# Autodesk Inventor assembly: ラックアンドピニオン
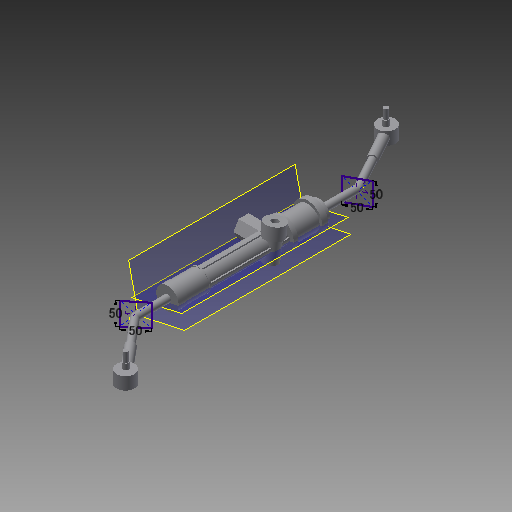
[picture p0: Inventor's stored thumbnail of the model, 512x512]
Saved by Autodesk Inventor 2018 (Build 220112000, 112)
## iProperties
Created: 2017-09-10
Part Number: ラックアンドピニオン
Material: 一般
Document SubType Name: Assembly
Designer: Kenta
Author: Kenta
## Documents named in this file (4)
- C:\Users\Kenta\Documents\workspace\rbbr\cart\ラックアンドピニオン.iam
- C:\Users\Kenta\Documents\workspace\rbbr\cart\らっくあんどぴにおん.ipt
- C:\Users\Kenta\Documents\workspace\rbbr\cart\ラックアンドピニオンの中心棒.ipt
- C:\Users\Kenta\Documents\workspace\rbbr\cart\ラックアンドピニオンの左右の棒.ipt
## Components (4 placed, 3 different names)
1. らっくあんどぴにおん:1 — メイト:1, メイト:2, メイト:3, メイト:4, 角度:3, メイト:5, 角度:4
2. ラックアンドピニオンの中心棒:1 — メイト:1, ボール:1, ボール:2
3. ラックアンドピニオンの左右の棒:1 — ボール:1
4. ラックアンドピニオンの左右の棒:2 — ボール:2
## Relationships (10: Mate 5, BallJoint 2, Angle 2, Flush 1)
- メイト:1 [Mate]: らっくあんどぴにおん:1 ↔ ラックアンドピニオンの中心棒:1
- ボール:1 [BallJoint]: ラックアンドピニオンの中心棒:1 ↔ ラックアンドピニオンの左右の棒:1
- ボール:2 [BallJoint]: ラックアンドピニオンの中心棒:1 ↔ ラックアンドピニオンの左右の棒:2
- メイト:2 [Mate]: らっくあんどぴにおん:1
- メイト:3 [Mate]: らっくあんどぴにおん:1
- メイト:4 [Mate]: らっくあんどぴにおん:1
- 角度:3 [Angle] (102.52 deg): らっくあんどぴにおん:1
- フラッシュ:1 [Flush] (30 mm)
- メイト:5 [Mate]: らっくあんどぴにおん:1
- 角度:4 [Angle] (12.52 deg): らっくあんどぴにおん:1
